# Autodesk Inventor assembly: mg996r_right_foot_frame
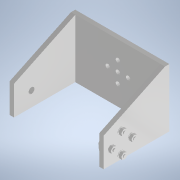
[picture p0: Inventor's stored thumbnail of the model, 180x180]
Saved by Autodesk Inventor 2021.4 (Build 254397000, 397)
## iProperties
Created: 2022-08-03
Part Number: mg996r_right_foot_frame
Document SubType Name: Assembly
Designer: isamu
Author: isamu
## Documents named in this file (6)
- D:\personal_projects\robot\inventor\2021_matlab_compat _v2\servo_rot_frame\mg996r_right_foot_frame.iam
- D:\personal_projects\robot\exports\frames\servo frame mg996 foot_MIR.ipt
- D:\personal_projects\robot\inventor\2021_matlab_compat _v2\servo_frames\servo_handle.iam
- D:\personal_projects\robot\exports\screws\m2 washer.ipt
- D:\personal_projects\robot\exports\screws\m2 nuts.ipt
- D:\personal_projects\robot\exports\screws\m4 nuts.ipt
## Components (11 placed, 5 different names)
1. servo frame mg996 foot_MIR:1 — Mate:1, Mate:2, Mate:3, Insert:1, Insert:2, Insert:3, Insert:4, Insert:6, Insert:9
2. servo_handle:1 [sub-assembly] — Mate:1, Mate:2, Mate:3
3. m2 washer:1 — Insert:1, Insert:5
4. m2 washer:2 — Insert:4, Insert:8
5. m2 washer:3 — Insert:2
6. m2 washer:4 — Insert:3, Insert:7
7. m2 nuts:1 — Insert:5
8. m2 nuts:2 — Insert:7
9. m2 nuts:3 — Insert:6
10. m2 nuts:4 — Insert:8
11. m4 nuts:1 — Insert:9
## Relationships (12: Insert 9, Mate 3)
- Mate:1: servo frame mg996 foot_MIR:1 ↔ servo_handle:1
- Mate:2: servo frame mg996 foot_MIR:1 ↔ servo_handle:1
- Mate:3: servo frame mg996 foot_MIR:1 ↔ servo_handle:1
- Insert:1: servo frame mg996 foot_MIR:1 ↔ m2 washer:1
- Insert:2: servo frame mg996 foot_MIR:1 ↔ m2 washer:3
- Insert:3: servo frame mg996 foot_MIR:1 ↔ m2 washer:4
- Insert:4: servo frame mg996 foot_MIR:1 ↔ m2 washer:2
- Insert:5: m2 washer:1 ↔ m2 nuts:1
- Insert:6: servo frame mg996 foot_MIR:1 ↔ m2 nuts:3
- Insert:7: m2 washer:4 ↔ m2 nuts:2
- Insert:8: m2 washer:2 ↔ m2 nuts:4
- Insert:9: servo frame mg996 foot_MIR:1 ↔ m4 nuts:1
